# Autodesk Inventor assembly: Trunk_neck_frame_AND_Trunk_shoulder_frame_WearingImage
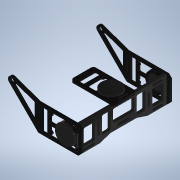
[picture p0: Inventor's stored thumbnail of the model, 180x180]
Saved by Autodesk Inventor 2022 (Build 260153000, 153)
## iProperties
Created: 2022-03-16
Part Number: Trunk_neck_frame_AND_Trunk_shoulder_frame_WearingImage
Document SubType Name: Assembly
Designer: Masato Kubotera
Author: Masato Kubotera
## iProperties of the stored document MemberDocs/xAaaaqbcaAaaaaaaaAaaaqxjcCb
Created: 2022-03-16
Part Number: Trunk_neck_frame_AND_Trunk_shoulder_frame_WearingImage
Document SubType Name: Assembly
Designer: Masato Kubotera
Author: Masato Kubotera
## Documents named in this file (6)
- C:\Users\Masato\Documents\Inventor\CIT Brains_Inventor\SUSTAINA-OP\OptionParts\SandBlastingJig\Trunk_neck_frame_AND_Trunk_shoulder_frame_WearingImage.iam
- C:\Users\Masato\Documents\Inventor\CIT Brains_Inventor\SUSTAINA-OP\UpperBody\Trunk\Trunk_neck_frame.ipt
- C:\Users\Masato\Documents\Inventor\CIT Brains_Inventor\SUSTAINA-OP\UpperBody\Trunk\Trunk_shoulder_frame_MIR.ipt
- C:\Users\Masato\Documents\Inventor\CIT Brains_Inventor\SUSTAINA-OP\OptionParts\SandBlastingJig\Trunk_neck_frame_AND_Trunk_shoulder_frame_SandBlastingJig.ipt
- C:\Users\Masato\Documents\Inventor\CIT Brains_Inventor\SUSTAINA-OP\UpperBody\Trunk\Trunk_shoulder_frame.ipt
- C:\Users\Masato\Documents\Inventor\CIT Brains_Inventor\SUSTAINA-OP\UpperBody\Trunk\Trunk_chest_frame.ipt
## Components (7 placed, 5 different names)
1. Trunk_neck_frame:1 — 挿入:2, フラッシュ:1, フラッシュ:2, フラッシュ:3, 挿入:5, 挿入:6
2. Trunk_shoulder_frame:1 — 挿入:3, 挿入:9, 挿入:10
3. Trunk_shoulder_frame_MIR:1 — 挿入:4, 挿入:7, 挿入:8
4. Trunk_neck_frame_AND_Trunk_shoulder_frame_SandBlastingJig:1 — 挿入:2
5. Trunk_neck_frame_AND_Trunk_shoulder_frame_SandBlastingJig:2 — 挿入:4
6. Trunk_neck_frame_AND_Trunk_shoulder_frame_SandBlastingJig:3 — 挿入:3
7. Trunk_chest_frame:1 — 挿入:5, 挿入:6, 挿入:7, 挿入:8, 挿入:9, 挿入:10
## Relationships (12: Insert 9, Flush 3)
- 挿入:2 [Insert]: Trunk_neck_frame:1 ↔ Trunk_neck_frame_AND_Trunk_shoulder_frame_SandBlastingJig:1
- 挿入:3 [Insert]: Trunk_shoulder_frame:1 ↔ Trunk_neck_frame_AND_Trunk_shoulder_frame_SandBlastingJig:3
- 挿入:4 [Insert]: Trunk_shoulder_frame_MIR:1 ↔ Trunk_neck_frame_AND_Trunk_shoulder_frame_SandBlastingJig:2
- フラッシュ:1 [Flush]: Trunk_neck_frame:1
- フラッシュ:2 [Flush]: Trunk_neck_frame:1
- フラッシュ:3 [Flush]: Trunk_neck_frame:1
- 挿入:5 [Insert]: Trunk_neck_frame:1 ↔ Trunk_chest_frame:1
- 挿入:6 [Insert]: Trunk_neck_frame:1 ↔ Trunk_chest_frame:1
- 挿入:7 [Insert]: Trunk_shoulder_frame_MIR:1 ↔ Trunk_chest_frame:1
- 挿入:8 [Insert]: Trunk_shoulder_frame_MIR:1 ↔ Trunk_chest_frame:1
- 挿入:9 [Insert]: Trunk_shoulder_frame:1 ↔ Trunk_chest_frame:1
- 挿入:10 [Insert]: Trunk_shoulder_frame:1 ↔ Trunk_chest_frame:1
